# Autodesk Inventor assembly: tower
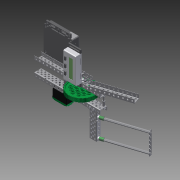
[picture p0: Inventor's stored thumbnail of the model, 180x180]
Saved by Autodesk Inventor 2014 SP1 (Build 180222100, 222)
## iProperties
Created: 2014-03-19
Part Number: tower
Document SubType Name: Assembly
Designer: Ryan
Author: Ryan
## Documents named in this file (26)
- C:\Users\Ryan\Desktop\sw\toss up 5th A bot\tower\tower.iam
- C:\Users\Ryan\Desktop\sw\lib\Aperture VEX CAD Library\Metal\C Channel\2 x 18.ipt
- C:\Users\Ryan\Desktop\sw\lib\Aperture VEX CAD Library\Bearing Blocks\Bearing Block.ipt
- C:\Users\Ryan\Desktop\sw\lib\Aperture VEX CAD Library\Hardware\8-32\8-32_.500.ipt
- C:\Users\Ryan\Desktop\sw\lib\Aperture VEX CAD Library\Hardware\8-32\8-32 nylock.ipt
- C:\Users\Ryan\Desktop\sw\lib\Aperture VEX CAD Library\Motors\2-Wire Motor 393-Without Wire.iam
- C:\Users\Ryan\Desktop\sw\lib\Aperture VEX CAD Library\Hardware\6-32\6-32_.250.ipt
- C:\Users\Ryan\Desktop\sw\lib\Aperture VEX CAD Library\Spacers\thin\SPACER-0320-0125.ipt
- C:\Users\Ryan\Desktop\sw\lib\Aperture VEX CAD Library\Gears\High Strength Gears\HS-GEAR-12TOOTH.ipt
- C:\Users\Ryan\Desktop\sw\lib\Aperture VEX CAD Library\Gears\High Strength Gears\Green HS 84.iam
- C:\Users\Ryan\Desktop\sw\lib\Aperture VEX CAD Library\Spacers\thin\SPACER-0320-0500.ipt
- C:\Users\Ryan\Desktop\sw\lib\Aperture VEX CAD Library\Spacers\thin\SPACER-0320-0250.ipt
- C:\Users\Ryan\Desktop\sw\lib\Aperture VEX CAD Library\Hardware\Shaft Collar.ipt
- C:\Users\Ryan\Desktop\sw\lib\Aperture VEX CAD Library\Spacers\thin\SPACER-0320-00625.ipt
- C:\Users\Ryan\Desktop\sw\lib\Aperture VEX CAD Library\Standoffs\BEAM-0500.ipt
- C:\Users\Ryan\Desktop\sw\toss up 5th A bot\tower\large ball knocker right.iam
- C:\Users\Ryan\Desktop\sw\lib\Aperture VEX CAD Library\Metal\L Bar\2 x 4.ipt
- C:\Users\Ryan\Desktop\sw\lib\Aperture VEX CAD Library\Hardware\8-32\8-32_.375.ipt
- C:\Users\Ryan\Desktop\sw\lib\Aperture VEX CAD Library\Hardware\8-32\8-32_1.500.ipt
- C:\Users\Ryan\Desktop\sw\lib\Aperture VEX CAD Library\Metal\Plate\2 x 5.ipt
- C:\Users\Ryan\Desktop\sw\lib\Aperture VEX CAD Library\Hardware\8-32\8-23_.750.ipt
- C:\Users\Ryan\Desktop\sw\lib\Aperture VEX CAD Library\Spacers\SPACER-0500-0125.ipt
- C:\Users\Ryan\Desktop\sw\lib\Aperture VEX CAD Library\Metal\C Channel\2 x 10.ipt
- C:\Users\Ryan\Desktop\sw\lib\Aperture VEX CAD Library\Spacers\thin\SPACER-0320-0375.ipt
- C:\Users\Ryan\Desktop\sw\lib\Super Sonic Sparks VEX CAD Library\Other Parts\(VEX) Cortex Microcontroller.iam
- C:\Users\Ryan\Desktop\sw\lib\Super Sonic Sparks VEX CAD Library\Other Parts\LCD Display.iam
## Components (74 placed, 25 different names)
1. 2 x 18:1 — Mate:1, Mate:3, Mate:4, Mate:5, Mate:6, Mate:7, Mate:8, Mate:9, Mate:10, Mate:11, Mate:12, Mate:13, Mate:15, Mate:17, Mate:26, Mate:33, Mate:34, Mate:35, Mate:36, Mate:37, Mate:39, Mate:46, Mate:48, Flush:6, Flush:7, Flush:8, Flush:9, Mate:87, Mate:91, Flush:11, Flush:12, Mate:92, Flush:13, Flush:14, Mate:134
2. Bearing Block:1 — Mate:1, Mate:3, Mate:4, Mate:5, Mate:14, Mate:16, Mate:18, Mate:21, Mate:71, Mate:88, Mate:93, Mate:94
3. Bearing Block:2 — Mate:6, Mate:7, Mate:8, Mate:9, Mate:22, Mate:23, Mate:31, Mate:32, Mate:40
4. Bearing Block:3 — Mate:10, Mate:11, Mate:12, Mate:13, Mate:24, Mate:25, Mate:38
5. 8-32_.500:1 — Mate:14, Mate:15, Mate:19
6. 8-32_.500:2 — Mate:16, Mate:17, Mate:20, Mate:74
7. 8-32 nylock:1 — Mate:18, Mate:19
8. 8-32 nylock:2 — Mate:20, Mate:21
9. 8-32_.500:3 — Mate:22, Flush:3, Mate:26, Mate:27
10. 8-32_.500:4 — Mate:23, Flush:2, Flush:3, Mate:28
11. 8-32_.500:5 — Mate:24, Flush:1, Flush:2, Mate:29
12. 8-32_.500:6 — Mate:25, Flush:1, Mate:30
13. 8-32 nylock:3 — Mate:27, Mate:31
14. 8-32 nylock:4 — Mate:28, Flush:4, Mate:80
15. 8-32 nylock:5 — Mate:29, Flush:4, Flush:5, Mate:32
16. 8-32 nylock:6 — Mate:30, Flush:5
17. 2-Wire Motor 393-Without Wire:1 [sub-assembly] — Mate:33, Mate:34, Mate:35, Mate:36, Mate:45, Mate:47
18. 6-32_.250:1 — Mate:45, Mate:46
19. SPACER-0320-0125:1 — Mate:37, Mate:38, Mate:41, Mate:42
20. SPACER-0320-0125:2 — Mate:39, Mate:40, Mate:43, Mate:44
21. HS-GEAR-12TOOTH:1 — Mate:41, Mate:42, Mate:49, Mate:50
22. Green HS 84:1 [sub-assembly] — Mate:43, Mate:44, Mate:51, Mate:76
23. 6-32_.250:2 — Mate:47, Mate:48
24. SPACER-0320-0500:1 — Mate:49, Mate:50, Mate:58
25. 2 x 18:2 — Flush:6, Flush:7, Flush:8, Mate:55, Mate:59, Mate:72, Mate:73, Mate:75, Mate:77, Mate:78, Mate:83, Mate:102, Flush:15, Flush:16, Mate:103, Mate:106, Mate:110, Mate:112, Mate:122, Mate:123, Mate:124, Mate:131, Mate:138, Mate:139, Mate:140, Mate:141, Mate:142, Mate:143, Mate:144, Angle:1, Mate:146, Mate:147, Mate:149
26. SPACER-0320-0250:1 — Mate:51, Mate:53, Mate:54, Mate:56, Mate:57
27. Shaft Collar:1 — Mate:53, Mate:54, Mate:55
28. SPACER-0320-00625:1 — Mate:56, Mate:57
29. Shaft Collar:2 — Mate:58, Mate:59
30. Bearing Block:4 — Mate:60, Mate:61, Mate:63, Mate:64, Mate:71, Mate:72, Mate:81, Mate:82, Mate:84
31. Bearing Block:5 — Mate:66, Mate:67, Mate:68, Mate:76, Mate:77, Mate:79
32. 8-32_.500:7 — Mate:60, Mate:62, Mate:75
33. 8-32_.500:8 — Mate:61, Mate:65, Mate:73, Mate:74
34. 8-32 nylock:7 — Mate:62, Mate:63
35. 8-32 nylock:8 — Mate:64, Mate:65
36. 8-32_.500:9 — Mate:66, Flush:10, Mate:69
37. 8-32_.500:10 — Flush:10, Mate:67, Mate:70, Mate:78
38. 8-32 nylock:9 — Mate:68, Mate:69
39. 8-32 nylock:10 — Mate:70, Mate:79, Mate:80
40. SPACER-0320-0125:3 — Mate:81, Mate:82, Mate:96
41. 8-32 nylock:11 — Mate:83, Mate:84, Mate:85, Mate:86
42. SPACER-0320-0125:4 — Mate:85, Mate:86, Mate:95
43. BEAM-0500:1 — Mate:87, Mate:88, Mate:89, Mate:90
44. SPACER-0320-0125:5 — Mate:89, Mate:90
45. large ball knocker right:1 [sub-assembly] — Mate:91, Flush:11, Flush:12, Angle:2
46. 2 x 4:1 — Mate:92, Flush:13, Flush:14, Mate:97, Mate:98, Mate:99, Mate:101, Mate:133, Mate:135
47. 8-32_.500:11 — Mate:93, Mate:94
48. 8-32_1.500:1 — Mate:95, Mate:96
49. 8-32 nylock:12 — Mate:97, Mate:98, Mate:99, Mate:100
50. 8-32_.375:1 — Mate:100, Mate:101
51. 2 x 5:1 — Mate:102, Flush:15, Flush:16, Mate:104, Mate:105, Mate:107, Mate:108, Mate:113, Mate:114, Mate:136
52. 8-32_.375:2 — Mate:103, Mate:104, Mate:105, Mate:111
53. 8-32_.375:3 — Mate:106, Mate:107, Mate:108, Mate:109
54. 8-32 nylock:13 — Mate:109, Mate:110
55. 8-32 nylock:14 — Mate:111, Mate:112
56. 8-23_.750:1 — Mate:113, Mate:114, Mate:115, Mate:116, Mate:117, Mate:118
57. BEAM-0500:2 — Mate:115, Mate:119, Mate:137
58. SPACER-0500-0125:1 — Mate:116, Mate:117, Mate:137
59. 8-32 nylock:15 — Mate:118, Mate:119, Mate:136
60. SPACER-0320-0375:1 — Mate:120, Mate:121, Mate:123, Mate:125, Mate:126, Mate:127, Mate:128
61. SPACER-0320-0250:2 — Mate:120, Mate:121, Mate:122, Mate:124, Mate:130
62. 2 x 10:1 — Mate:125, Mate:126, Mate:127, Mate:129, Angle:2
63. 8-32_.375:4 — Mate:128, Mate:129
64. 8-32 nylock:16 — Mate:130, Mate:131
65. (VEX) Cortex Microcontroller:1 [sub-assembly] — Mate:138, Mate:139, Mate:140, Mate:141
66. LCD Display:1 [sub-assembly] — Mate:142, Mate:143, Mate:144, Angle:1, Mate:145
67. 8-32 nylock:17 — Mate:135
68. 8-32_.375:5 — Mate:133, Mate:134
69. 8-32 nylock:18
70. 8-32_.375:6
71. 8-32_.500:12 — Mate:145, Mate:146, Mate:147, Mate:148
72. 8-32 nylock:19 — Mate:148, Mate:149
73. 8-32_.500:13
74. 8-32 nylock:20
## Component patterns: (2 elements, first: 8-32 nylock:17 + 8-32_.375:5), (2 elements, first: 8-32_.500:12 + 8-32 nylock:19)
## Relationships (165: Mate 147, Flush 16, Angle 2)
- Mate:1: 2 x 18:1 ↔ Bearing Block:1
- Mate:3 (2.3114 mm): 2 x 18:1 ↔ Bearing Block:1
- Mate:4 (2.3114 mm): 2 x 18:1 ↔ Bearing Block:1
- Mate:5 (2.3114 mm): 2 x 18:1 ↔ Bearing Block:1
- Mate:6: 2 x 18:1 ↔ Bearing Block:2
- Mate:7 (2.3114 mm): 2 x 18:1 ↔ Bearing Block:2
- Mate:8 (2.3114 mm): 2 x 18:1 ↔ Bearing Block:2
- Mate:9 (2.3114 mm): 2 x 18:1 ↔ Bearing Block:2
- Mate:10 (2.3114 mm): 2 x 18:1 ↔ Bearing Block:3
- Mate:11: 2 x 18:1 ↔ Bearing Block:3
- Mate:12 (2.3114 mm): 2 x 18:1 ↔ Bearing Block:3
- Mate:13 (2.3114 mm): 2 x 18:1 ↔ Bearing Block:3
- Mate:14: Bearing Block:1 ↔ 8-32_.500:1
- Mate:15: 2 x 18:1 ↔ 8-32_.500:1
- Mate:16: Bearing Block:1 ↔ 8-32_.500:2
- Mate:17: 2 x 18:1 ↔ 8-32_.500:2
- Mate:18: Bearing Block:1 ↔ 8-32 nylock:1
- Mate:19: 8-32_.500:1 ↔ 8-32 nylock:1
- Mate:20: 8-32_.500:2 ↔ 8-32 nylock:2
- Mate:21: Bearing Block:1 ↔ 8-32 nylock:2
- Mate:22: Bearing Block:2 ↔ 8-32_.500:3
- Mate:23: Bearing Block:2 ↔ 8-32_.500:4
- Mate:24: Bearing Block:3 ↔ 8-32_.500:5
- Mate:25: Bearing Block:3 ↔ 8-32_.500:6
- Flush:1: 8-32_.500:5 ↔ 8-32_.500:6
- Flush:2: 8-32_.500:4 ↔ 8-32_.500:5
- Flush:3: 8-32_.500:3 ↔ 8-32_.500:4
- Mate:26: 2 x 18:1 ↔ 8-32_.500:3
- Mate:27: 8-32_.500:3 ↔ 8-32 nylock:3
- Mate:28: 8-32_.500:4 ↔ 8-32 nylock:4
- Mate:29: 8-32_.500:5 ↔ 8-32 nylock:5
- Mate:30: 8-32_.500:6 ↔ 8-32 nylock:6
- Mate:31: Bearing Block:2 ↔ 8-32 nylock:3
- Flush:4: 8-32 nylock:4 ↔ 8-32 nylock:5
- Flush:5: 8-32 nylock:5 ↔ 8-32 nylock:6
- Mate:32: Bearing Block:2 ↔ 8-32 nylock:5
- Mate:33: 2 x 18:1 ↔ 2-Wire Motor 393-Without Wire:1
- Mate:34 (2.3114 mm): 2 x 18:1 ↔ 2-Wire Motor 393-Without Wire:1
- Mate:35 (2.3114 mm): 2 x 18:1 ↔ 2-Wire Motor 393-Without Wire:1
- Mate:36 (2.3114 mm): 2 x 18:1 ↔ 2-Wire Motor 393-Without Wire:1
- Mate:37: 2 x 18:1 ↔ SPACER-0320-0125:1
- Mate:38: Bearing Block:3 ↔ SPACER-0320-0125:1
- Mate:39: 2 x 18:1 ↔ SPACER-0320-0125:2
- Mate:40: Bearing Block:2 ↔ SPACER-0320-0125:2
- Mate:41: SPACER-0320-0125:1 ↔ HS-GEAR-12TOOTH:1
- Mate:42: SPACER-0320-0125:1 ↔ HS-GEAR-12TOOTH:1
- Mate:43: SPACER-0320-0125:2 ↔ Green HS 84:1
- Mate:44: SPACER-0320-0125:2 ↔ Green HS 84:1
- Mate:45: 2-Wire Motor 393-Without Wire:1 ↔ 6-32_.250:1
- Mate:46: 2 x 18:1 ↔ 6-32_.250:1
- Mate:47: 2-Wire Motor 393-Without Wire:1 ↔ 6-32_.250:2
- Mate:48: 2 x 18:1 ↔ 6-32_.250:2
- Mate:49: HS-GEAR-12TOOTH:1 ↔ SPACER-0320-0500:1
- Mate:50: HS-GEAR-12TOOTH:1 ↔ SPACER-0320-0500:1
- Flush:6: 2 x 18:1 ↔ 2 x 18:2
- Flush:7: 2 x 18:1 ↔ 2 x 18:2
- Flush:8 (50.8 mm): 2 x 18:1 ↔ 2 x 18:2
- Mate:51: Green HS 84:1 ↔ SPACER-0320-0250:1
- Mate:53: SPACER-0320-0250:1 ↔ Shaft Collar:1
- Mate:54: SPACER-0320-0250:1 ↔ Shaft Collar:1
- Mate:55: 2 x 18:2 ↔ Shaft Collar:1
- Mate:56: SPACER-0320-0250:1 ↔ SPACER-0320-00625:1
- Mate:57: SPACER-0320-0250:1 ↔ SPACER-0320-00625:1
- Mate:58: SPACER-0320-0500:1 ↔ Shaft Collar:2
- Mate:59: 2 x 18:2 ↔ Shaft Collar:2
- Flush:9 (17.8816 mm): 2 x 18:1
- Mate:60: Bearing Block:4 ↔ 8-32_.500:7
- Mate:61: Bearing Block:4 ↔ 8-32_.500:8
- Mate:62: 8-32_.500:7 ↔ 8-32 nylock:7
- Mate:63: Bearing Block:4 ↔ 8-32 nylock:7
- Mate:64: Bearing Block:4 ↔ 8-32 nylock:8
- Mate:65: 8-32_.500:8 ↔ 8-32 nylock:8
- Mate:66: Bearing Block:5 ↔ 8-32_.500:9
- Flush:10: 8-32_.500:9 ↔ 8-32_.500:10
- Mate:67: Bearing Block:5 ↔ 8-32_.500:10
- Mate:68: Bearing Block:5 ↔ 8-32 nylock:9
- Mate:69: 8-32_.500:9 ↔ 8-32 nylock:9
- Mate:70: 8-32_.500:10 ↔ 8-32 nylock:10
- Mate:71: Bearing Block:1 ↔ Bearing Block:4
- Mate:72: 2 x 18:2 ↔ Bearing Block:4
- Mate:73: 2 x 18:2 ↔ 8-32_.500:8
- Mate:74: 8-32_.500:2 ↔ 8-32_.500:8
- Mate:75: 2 x 18:2 ↔ 8-32_.500:7
- Mate:76: Green HS 84:1 ↔ Bearing Block:5
- Mate:77: 2 x 18:2 ↔ Bearing Block:5
- Mate:78: 2 x 18:2 ↔ 8-32_.500:10
- Mate:79: Bearing Block:5 ↔ 8-32 nylock:10
- Mate:80: 8-32 nylock:4 ↔ 8-32 nylock:10
- Mate:81: Bearing Block:4 ↔ SPACER-0320-0125:3
- Mate:82: Bearing Block:4 ↔ SPACER-0320-0125:3
- Mate:83: 2 x 18:2 ↔ 8-32 nylock:11
- Mate:84: Bearing Block:4 ↔ 8-32 nylock:11
- Mate:85: 8-32 nylock:11 ↔ SPACER-0320-0125:4
- Mate:86: 8-32 nylock:11 ↔ SPACER-0320-0125:4
- Mate:87: 2 x 18:1 ↔ BEAM-0500:1
- Mate:88: Bearing Block:1 ↔ BEAM-0500:1
- Mate:89: BEAM-0500:1 ↔ SPACER-0320-0125:5
- Mate:90: BEAM-0500:1 ↔ SPACER-0320-0125:5
- Mate:91: 2 x 18:1 ↔ large ball knocker right:1
- Flush:11: 2 x 18:1 ↔ large ball knocker right:1
- Flush:12: 2 x 18:1 ↔ large ball knocker right:1
- Mate:92: 2 x 18:1 ↔ 2 x 4:1
- Flush:13: 2 x 18:1 ↔ 2 x 4:1
- Flush:14: 2 x 18:1 ↔ 2 x 4:1
- Mate:93: Bearing Block:1 ↔ 8-32_.500:11
- Mate:94: Bearing Block:1 ↔ 8-32_.500:11
- Mate:95: SPACER-0320-0125:4 ↔ 8-32_1.500:1
- Mate:96: SPACER-0320-0125:3 ↔ 8-32_1.500:1
- Mate:97 (1.1684 mm): 2 x 4:1 ↔ 8-32 nylock:12
- Mate:98 (2.3114 mm): 2 x 4:1 ↔ 8-32 nylock:12
- Mate:99 (2.3114 mm): 2 x 4:1 ↔ 8-32 nylock:12
- Mate:100: 8-32 nylock:12 ↔ 8-32_.375:1
- Mate:101: 2 x 4:1 ↔ 8-32_.375:1
- Mate:102: 2 x 18:2 ↔ 2 x 5:1
- Flush:15: 2 x 18:2 ↔ 2 x 5:1
- Flush:16: 2 x 18:2 ↔ 2 x 5:1
- Mate:103 (2.3114 mm): 2 x 18:2 ↔ 8-32_.375:2
- Mate:104 (2.3114 mm): 2 x 5:1 ↔ 8-32_.375:2
- Mate:105: 2 x 5:1 ↔ 8-32_.375:2
- Mate:106 (2.3114 mm): 2 x 18:2 ↔ 8-32_.375:3
- Mate:107 (2.3114 mm): 2 x 5:1 ↔ 8-32_.375:3
- Mate:108: 2 x 5:1 ↔ 8-32_.375:3
- Mate:109: 8-32_.375:3 ↔ 8-32 nylock:13
- Mate:110: 2 x 18:2 ↔ 8-32 nylock:13
- Mate:111: 8-32_.375:2 ↔ 8-32 nylock:14
- Mate:112: 2 x 18:2 ↔ 8-32 nylock:14
- Mate:113 (2.3114 mm): 2 x 5:1 ↔ 8-23_.750:1
- Mate:114 (2.3114 mm): 2 x 5:1 ↔ 8-23_.750:1
- Mate:115: 8-23_.750:1 ↔ BEAM-0500:2
- Mate:116: 8-23_.750:1 ↔ SPACER-0500-0125:1
- Mate:117: 8-23_.750:1 ↔ SPACER-0500-0125:1
- Mate:118: 8-23_.750:1 ↔ 8-32 nylock:15
- Mate:119 (1.1684 mm): BEAM-0500:2 ↔ 8-32 nylock:15
- Mate:120: SPACER-0320-0375:1 ↔ SPACER-0320-0250:2
- Mate:121: SPACER-0320-0375:1 ↔ SPACER-0320-0250:2
- Mate:122: 2 x 18:2 ↔ SPACER-0320-0250:2
- Mate:123 (2.3114 mm): 2 x 18:2 ↔ SPACER-0320-0375:1
- Mate:124 (2.3114 mm): 2 x 18:2 ↔ SPACER-0320-0250:2
- Mate:125: SPACER-0320-0375:1 ↔ 2 x 10:1
- Mate:126 (2.3114 mm): SPACER-0320-0375:1 ↔ 2 x 10:1
- Mate:127 (2.3114 mm): SPACER-0320-0375:1 ↔ 2 x 10:1
- Mate:128: SPACER-0320-0375:1 ↔ 8-32_.375:4
- Mate:129: 2 x 10:1 ↔ 8-32_.375:4
- Mate:130: SPACER-0320-0250:2 ↔ 8-32 nylock:16
- Mate:131: 2 x 18:2 ↔ 8-32 nylock:16
- [Mate]: 8-32 nylock:17 ↔ 8-32_.375:5
- Mate:133 (2.3114 mm): 2 x 4:1 ↔ 8-32_.375:5
- Mate:134: 2 x 18:1 ↔ 8-32_.375:5
- Mate:135: 2 x 4:1 ↔ 8-32 nylock:17
- Mate:136: 2 x 5:1 ↔ 8-32 nylock:15
- Mate:137: BEAM-0500:2 ↔ SPACER-0500-0125:1
- Mate:138: 2 x 18:2 ↔ (VEX) Cortex Microcontroller:1
- Mate:139 (2.3114 mm): 2 x 18:2 ↔ (VEX) Cortex Microcontroller:1
- Mate:140 (2.3114 mm): 2 x 18:2 ↔ (VEX) Cortex Microcontroller:1
- Mate:141 (2.3114 mm): 2 x 18:2 ↔ (VEX) Cortex Microcontroller:1
- Mate:142: 2 x 18:2 ↔ LCD Display:1
- Mate:143 (2.3114 mm): 2 x 18:2 ↔ LCD Display:1
- Mate:144 (2.3114 mm): 2 x 18:2 ↔ LCD Display:1
- Angle:1 (90 deg): 2 x 18:2 ↔ LCD Display:1
- Mate:145: LCD Display:1 ↔ 8-32_.500:12
- Mate:146 (2.3114 mm): 2 x 18:2 ↔ 8-32_.500:12
- Mate:147 (2.3114 mm): 2 x 18:2 ↔ 8-32_.500:12
- Mate:148: 8-32_.500:12 ↔ 8-32 nylock:19
- Mate:149: 2 x 18:2 ↔ 8-32 nylock:19
- Angle:2 (-90 deg): large ball knocker right:1 ↔ 2 x 10:1
## Named parameters: q = 2.3114 mm, d148_d114 = 0 mm
